# Autodesk Inventor assembly: Ellbow
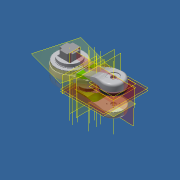
[picture p0: Inventor's stored thumbnail of the model, 180x180]
Saved by Autodesk Inventor 2016 (Build 200138000, 138)
## iProperties
Created: 2015-08-24
Part Number: Ellbow
Material: Generisch
Document SubType Name: Assembly
Designer: 4ndreas
Author: 4ndreas
## Documents named in this file (8)
- C:\Users\4ndreas\Documents\Inventor\RobotARM v2\v4\Ellbow.iam
- C:\Users\4ndreas\Documents\Inventor\RobotARM v2\v4\Ellbow\Konstruktions-Assistent\Übertragung des Zahnriemens1.iam
- C:\Users\4ndreas\Documents\Inventor\RobotARM v2\v4\Nema24.ipt
- C:\Users\4ndreas\Documents\Inventor\RobotARM v2\v4\Ellbow\Konstruktions-Assistent\Übertragung des Zahnriemens2.iam
- C:\Users\4ndreas\Documents\Inventor\RobotARM v2\v4\Joint_A_gear_Nema24.ipt
- C:\Users\4ndreas\Documents\Inventor\RobotARM v2\v4\Ellbow_bearing N24.ipt
- C:\Users\4ndreas\Documents\Inventor\RobotARM v2\v4\Joint_A N24.ipt
- C:\Users\4ndreas\Documents\Inventor\RobotARM v2\v2\encoder.iam
## Components (7 placed, 6 different names)
1. Ellbow_bearing N24:1 — Passend:1, Passend:2, Fluchtend:1, Passend:5, Winkel:1, Passend:8, Fluchtend:2, Passend:17, Passend:18
2. Übertragung des Zahnriemens:1 [sub-assembly] — Passend:16
3. Nema24:1 — Passend:3, Passend:7, Winkel:1, Passend:9, Passend:10, Passend:11
4. Übertragung des Zahnriemens:2 [sub-assembly] — Passend:15
5. Joint_A_gear_Nema24:1 — Passend:5, Passend:7, Passend:8, Passend:9, Passend:14, Fluchtend:3
6. Joint_A N24:1 — Passend:14, Passend:15, Fluchtend:3
7. encoder:1 [sub-assembly] — Passend:16, Passend:17, Passend:18
## Relationships (20: Mate 16, Flush 3, Angle 1)
- Passend:1 [Mate]: Ellbow_bearing N24:1
- Passend:2 [Mate]: Ellbow_bearing N24:1
- Fluchtend:1 [Flush] (70 mm): Ellbow_bearing N24:1
- Passend:3 [Mate]: Nema24:1
- Passend:5 [Mate]: Ellbow_bearing N24:1 ↔ Joint_A_gear_Nema24:1
- Passend:7 [Mate]: Nema24:1 ↔ Joint_A_gear_Nema24:1
- Winkel:1 [Angle] (0 deg): Ellbow_bearing N24:1 ↔ Nema24:1
- Passend:8 [Mate]: Ellbow_bearing N24:1 ↔ Joint_A_gear_Nema24:1
- Passend:9 [Mate]: Nema24:1 ↔ Joint_A_gear_Nema24:1
- Passend:10 [Mate]: Nema24:1
- Passend:11 [Mate]: Nema24:1
- Passend:12 [Mate]
- Passend:13 [Mate]
- Fluchtend:2 [Flush] (40 mm): Ellbow_bearing N24:1
- Passend:14 [Mate]: Joint_A_gear_Nema24:1 ↔ Joint_A N24:1
- Passend:15 [Mate]: Übertragung des Zahnriemens:2 ↔ Joint_A N24:1
- Fluchtend:3 [Flush]: Joint_A_gear_Nema24:1 ↔ Joint_A N24:1
- Passend:16 [Mate]: Übertragung des Zahnriemens:1 ↔ encoder:1
- Passend:17 [Mate]: Ellbow_bearing N24:1 ↔ encoder:1
- Passend:18 [Mate]: Ellbow_bearing N24:1 ↔ encoder:1
